# Autodesk Inventor assembly: splitter1
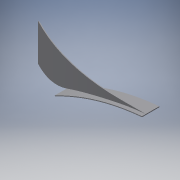
[picture p0: Inventor's stored thumbnail of the model, 180x180]
Saved by Autodesk Inventor 2018 (Build 220112000, 112)
## iProperties
Created: 2018-06-13
Part Number: splitter1
Material: 一般
Document SubType Name: Assembly
Designer: ku_sk
Author: ku_sk
## Documents named in this file (3)
- Z:\各班フォルダ\2018\ボディ\エアロ\Aero\KS-15\コスト用CAD\Frwing\parts\splitter1.iam
- Z:\各班フォルダ\2018\ボディ\エアロ\Aero\KS-15\コスト用CAD\Frwing\parts\Part11.ipt
- Z:\各班フォルダ\2018\ボディ\エアロ\Aero\KS-15\コスト用CAD\Frwing\parts\Part21.ipt
## Components (2 placed, 2 different names)
1. Part11:1 — メイト:1, 角度:1
2. Part21:1
## Relationships (2: Mate 1, Angle 1)
- メイト:1 [Mate]: Part11:1
- 角度:1 [Angle] (0 deg): Part11:1
